# Autodesk Inventor assembly: Full Box
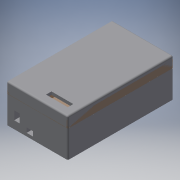
[picture p0: Inventor's stored thumbnail of the model, 180x180]
Saved by Autodesk Inventor 2019.3 (Build 233278000, 278)
## iProperties
Created: 2019-04-10
Part Number: Full Box
Document SubType Name: Assembly
Designer: grego
Author: grego
## Documents named in this file (3)
- D:\OneDrive - njit.edu\ECE 414-001\CAD model\Full Box.iam
- D:\OneDrive - njit.edu\ECE 414-001\CAD model\Smart Lock Box.ipt
- D:\OneDrive - njit.edu\ECE 414-001\CAD model\Smart Lock Box Top.ipt
## Components (2 placed, 2 different names)
1. Smart Lock Box:1 — Flush:1, Flush:2, Mate:1
2. Smart Lock Box Top:1 — Flush:1, Flush:2, Mate:1
## Relationships (3: Flush 2, Mate 1)
- Flush:1: Smart Lock Box:1 ↔ Smart Lock Box Top:1
- Flush:2: Smart Lock Box:1 ↔ Smart Lock Box Top:1
- Mate:1: Smart Lock Box:1 ↔ Smart Lock Box Top:1
